# Autodesk Inventor assembly: iris
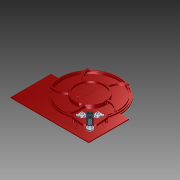
[picture p0: Inventor's stored thumbnail of the model, 180x180]
Saved by Autodesk Inventor 2015 (Build 190159000, 159)
## iProperties
Created: 2015-02-04
Part Number: iris
Document SubType Name: Assembly
Designer: janov_000
Author: janov_000
## Documents named in this file (12)
- C:\Users\janov_000\Documents\EiT iris\iris.iam
- C:\Users\janov_000\Documents\EiT iris\bakplate.ipt
- C:\Users\janov_000\Documents\EiT iris\ytterring.ipt
- C:\Users\janov_000\Documents\EiT iris\blad.ipt
- C:\Users\janov_000\Documents\EiT iris\ledeplate.ipt
- C:\Users\janov_000\Documents\EiT iris\MBR18_2_N8.ipt
- C:\Users\janov_000\Documents\EiT iris\AX12\AX12.iam
- C:\Users\janov_000\Documents\EiT iris\HBR8.iam
- C:\Users\janov_000\Documents\EiT iris\avstandsstykke.ipt
- C:\Users\janov_000\Documents\EiT iris\motorplate.ipt
- C:\Users\janov_000\Documents\EiT iris\innerring.ipt
- C:\Users\janov_000\Documents\EiT iris\motor_trinse.ipt
## Components (24 placed, 11 different names)
1. bakplate:1 — Mate:2, Insert:1, Mate:3, Insert:2, Rotational:1, Insert:7, Insert:10, Insert:11, Insert:16, Insert:18, Insert:19, Insert:22
2. ytterring:1 — Flush:1, Insert:3, Rotational:1, Insert:6, Insert:9, Insert:12, Insert:13
3. blad:1 — Mate:2, Insert:1, Insert:4
4. blad:2 — Mate:3, Insert:2, Insert:5, Mate:14, Insert:37
5. ledeplate:1 — Flush:1, Insert:3, Insert:4
6. ledeplate:2 — Insert:5, Insert:6
7. blad:3 — Insert:7, Insert:8
8. ledeplate:3 — Insert:8, Insert:9
9. blad:4 — Insert:10, Insert:14
10. blad:5 — Insert:11, Insert:15, Insert:36
11. ledeplate:4 — Insert:12, Insert:14
12. ledeplate:5 — Insert:13, Insert:15
13. MBR18-2-N8:1 — Insert:31
14. MBR18-2-N8:2 — Insert:30
15. AX12:1 [sub-assembly] — Mate:10, Mate:12, Mate:13, Insert:40
16. HBR8:1 [sub-assembly] — Mate:7, Insert:32, Insert:34
17. HBR8:2 [sub-assembly] — Mate:6, Insert:33, Insert:35
18. avstandsstykke:1 — Insert:16, Insert:17, Insert:22, Insert:23
19. avstandsstykke:2 — Insert:17, Insert:23, Insert:38
20. avstandsstykke:3 — Insert:18, Insert:19, Insert:20, Insert:21
21. avstandsstykke:4 — Insert:20, Insert:21, Insert:39
22. motorplate:1 — Mate:6, Mate:7, Insert:30, Insert:31, Insert:32, Insert:33, Insert:34, Insert:35, Mate:10, Mate:12, Mate:13, Insert:38, Insert:39
23. innerring:1 — Mate:14, Insert:36, Insert:37
24. motor_trinse:1 — Insert:40
## Relationships (44: Insert 34, Mate 8, Flush 1, RevoluteJoint 1)
- Mate:2: bakplate:1 ↔ blad:1
- Insert:1: bakplate:1 ↔ blad:1
- Mate:3: bakplate:1 ↔ blad:2
- Insert:2: bakplate:1 ↔ blad:2
- Flush:1: ytterring:1 ↔ ledeplate:1
- Insert:3: ytterring:1 ↔ ledeplate:1
- Insert:4: blad:1 ↔ ledeplate:1
- Rotational:1 [RevoluteJoint]: bakplate:1 ↔ ytterring:1
- Insert:5: blad:2 ↔ ledeplate:2
- Insert:6: ytterring:1 ↔ ledeplate:2
- Insert:7: bakplate:1 ↔ blad:3
- Insert:8: blad:3 ↔ ledeplate:3
- Insert:9: ytterring:1 ↔ ledeplate:3
- Insert:10: bakplate:1 ↔ blad:4
- Insert:11: bakplate:1 ↔ blad:5
- Insert:12: ytterring:1 ↔ ledeplate:4
- Insert:13: ytterring:1 ↔ ledeplate:5
- Insert:14: blad:4 ↔ ledeplate:4
- Insert:15: blad:5 ↔ ledeplate:5
- Insert:16: bakplate:1 ↔ avstandsstykke:1
- Insert:17: avstandsstykke:1 ↔ avstandsstykke:2
- Insert:18: bakplate:1 ↔ avstandsstykke:3
- Insert:19: bakplate:1 ↔ avstandsstykke:3
- Insert:20: avstandsstykke:3 ↔ avstandsstykke:4
- Insert:21: avstandsstykke:3 ↔ avstandsstykke:4
- Insert:22: bakplate:1 ↔ avstandsstykke:1
- Insert:23: avstandsstykke:1 ↔ avstandsstykke:2
- Mate:6: HBR8:2 ↔ motorplate:1
- Mate:7: HBR8:1 ↔ motorplate:1
- Insert:30 (1.5 mm): MBR18-2-N8:2 ↔ motorplate:1
- Insert:31 (1.5 mm): MBR18-2-N8:1 ↔ motorplate:1
- Insert:32: HBR8:1 ↔ motorplate:1
- Insert:33: HBR8:2 ↔ motorplate:1
- Insert:34: HBR8:1 ↔ motorplate:1
- Insert:35: HBR8:2 ↔ motorplate:1
- Mate:10: AX12:1 ↔ motorplate:1
- Mate:12 (1.5 mm): AX12:1 ↔ motorplate:1
- Mate:13 (1.5 mm): AX12:1 ↔ motorplate:1
- Mate:14: blad:2 ↔ innerring:1
- Insert:36: blad:5 ↔ innerring:1
- Insert:37: blad:2 ↔ innerring:1
- Insert:38: avstandsstykke:2 ↔ motorplate:1
- Insert:39: avstandsstykke:4 ↔ motorplate:1
- Insert:40: AX12:1 ↔ motor_trinse:1
